# Autodesk Inventor assembly: Сборка ручка
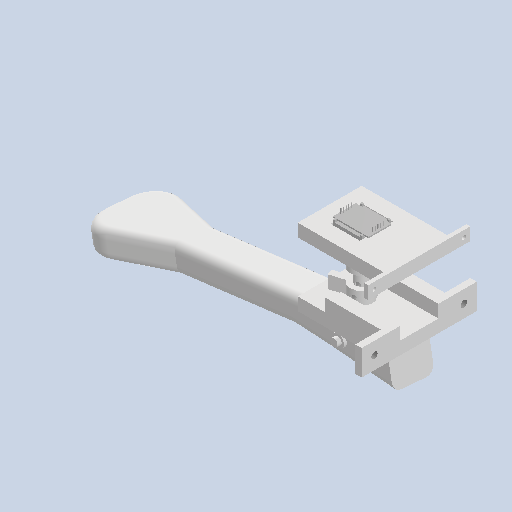
[picture p0: Inventor's stored thumbnail of the model, 512x512]
Saved by Autodesk Inventor 2023 (Build 270158000, 158)
## iProperties
Created: 2022-05-02
Part Number: Сборка ручка
Document SubType Name: Assembly
Designer: User
Author: User
## Documents named in this file (12)
- D:\Стойка\VR-simulator-3D-models\Механизм ручки\Сборка ручка.iam
- D:\Стойка\VR-simulator-3D-models\Механизм ручки\EAW.ipt
- D:\Стойка\VR-simulator-3D-models\Механизм ручки\Вал ручки.ipt
- D:\Стойка\VR-simulator-3D-models\Механизм ручки\Втулка энкодер.ipt
- D:\Стойка\VR-simulator-3D-models\Механизм ручки\Ручка.ipt
- D:\Стойка\VR-simulator-3D-models\Механизм ручки\Стенка.ipt
- D:\Стойка\VR-simulator-3D-models\Механизм ручки\Стопор.ipt
- D:\Стойка\VR-simulator-3D-models\Механизм ручки\Стенка энкодер.ipt
- D:\Стойка\VR-simulator-3D-models\Механизм ручки\Диск.ipt
- D:\Стойка\VR-simulator-3D-models\Механизм ручки\М3х8.ipt
- D:\Стойка\VR-simulator-3D-models\Механизм ручки\Шпилька.ipt
- D:\Стойка\VR-simulator-3D-models\Механизм ручки\Диск конец вала.ipt
## Components (14 placed, 11 different names)
1. EAW:1 — Цилиндрический:4, Совмещение:15, Совмещение:18
2. Вал ручки:1 — Цилиндрический:12, Цилиндрический:13, Совмещение:13, Цилиндрический:14, Цилиндрический:15, Совмещение:19
3. Втулка энкодер:1 — Цилиндрический:4, Цилиндрический:15, Совмещение:19, Совмещение:20
4. Ручка:1 — Совмещение:4, Совмещение:5, Цилиндрический:12, Совмещение:11, Совмещение:12
5. Стенка:1 — Заподлицо:1, Заподлицо:2, Совмещение:4, Цилиндрический:14, Совмещение:14
6. Стопор:1 — Цилиндрический:13, Совмещение:13, Совмещение:14
7. Стенка энкодер:1 — Заподлицо:1, Заподлицо:2, Совмещение:15, Совмещение:18, Совмещение:20
8. М3х8:1 — Цилиндрический:11, Совмещение:6
9. Диск:2 — Цилиндрический:10, Совмещение:7, Совмещение:8
10. М3х8:2 — Цилиндрический:9, Цилиндрический:10, Совмещение:7
11. Диск:3 — Цилиндрический:8, Совмещение:9, Совмещение:10, Совмещение:11
12. М3х8:3 — Цилиндрический:7, Цилиндрический:8, Совмещение:10, Совмещение:12
13. Шпилька:1 — Цилиндрический:7, Цилиндрический:9, Совмещение:8, Совмещение:9
14. Диск конец вала:1 — Цилиндрический:11, Совмещение:5, Совмещение:6
## Relationships (27: Mate 15, CylindricalJoint 10, Flush 2)
- Заподлицо:1 [Flush]: Стенка:1 ↔ Стенка энкодер:1
- Цилиндрический:4 [CylindricalJoint]: EAW:1 ↔ Втулка энкодер:1
- Заподлицо:2 [Flush]: Стенка:1 ↔ Стенка энкодер:1
- Цилиндрический:7 [CylindricalJoint]: М3х8:3 ↔ Шпилька:1
- Цилиндрический:8 [CylindricalJoint]: Диск:3 ↔ М3х8:3
- Цилиндрический:9 [CylindricalJoint]: М3х8:2 ↔ Шпилька:1
- Цилиндрический:10 [CylindricalJoint]: Диск:2 ↔ М3х8:2
- Цилиндрический:11 [CylindricalJoint]: М3х8:1 ↔ Диск конец вала:1
- Совмещение:4 [Mate]: Ручка:1 ↔ Стенка:1
- Совмещение:5 [Mate]: Ручка:1 ↔ Диск конец вала:1
- Совмещение:6 [Mate]: М3х8:1 ↔ Диск конец вала:1
- Цилиндрический:12 [CylindricalJoint]: Вал ручки:1 ↔ Ручка:1
- Совмещение:7 [Mate]: Диск:2 ↔ М3х8:2
- Совмещение:8 [Mate]: Диск:2 ↔ Шпилька:1
- Совмещение:9 [Mate]: Диск:3 ↔ Шпилька:1
- Совмещение:10 [Mate]: Диск:3 ↔ М3х8:3
- Совмещение:11 [Mate]: Ручка:1 ↔ Диск:3
- Совмещение:12 [Mate]: Ручка:1 ↔ М3х8:3
- Цилиндрический:13 [CylindricalJoint]: Вал ручки:1 ↔ Стопор:1
- Совмещение:13 [Mate]: Вал ручки:1 ↔ Стопор:1
- Цилиндрический:14 [CylindricalJoint]: Вал ручки:1 ↔ Стенка:1
- Совмещение:14 [Mate]: Стенка:1 ↔ Стопор:1
- Совмещение:15 [Mate]: EAW:1 ↔ Стенка энкодер:1
- Совмещение:18 [Mate]: EAW:1 ↔ Стенка энкодер:1
- Цилиндрический:15 [CylindricalJoint]: Вал ручки:1 ↔ Втулка энкодер:1
- Совмещение:19 [Mate]: Вал ручки:1 ↔ Втулка энкодер:1
- Совмещение:20 [Mate]: Втулка энкодер:1 ↔ Стенка энкодер:1
